# Autodesk Inventor assembly: Robot mrk3
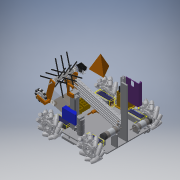
[picture p0: Inventor's stored thumbnail of the model, 180x180]
Saved by Autodesk Inventor 2019 (Build 230136000, 136)
## iProperties
Created: 2017-12-06
Part Number: Robot mrk3
Document SubType Name: Assembly
Designer: User
Author: User
## Documents named in this file (21)
- C:\Robotics\CAD\2018-19_CAD\Robot mrk2.iam
- C:\Robotics\CAD\2017-18_CAD\Prototypes\Gen2PlatePart.ipt
- C:\Robotics\CAD\2017-18_CAD\Prototypes\MecanumWheelFullForVexmotor.iam
- C:\Robotics\CAD\COTSParts\Rev\REV-41-1300HexMotor.ipt
- C:\Robotics\CAD\2017-18_CAD\Prototypes\MotorHolderA.ipt
- C:\Robotics\CAD\2017-18_CAD\Prototypes\MotorHolderB.ipt
- C:\Robotics\CAD\2018-19_CAD\Collection\20X20 lift.iam
- C:\Robotics\CAD\2018-19_CAD\Collection\SlidesPivotBracket.ipt
- C:\Robotics\CAD\2018-19_CAD\Collection\PaddleCollection2.1.ipt.iam
- C:\Robotics\CAD\2018-19_CAD\lift\lift assembly\Lead Screw Prototype A.iam
- C:\Robotics\CAD\2018-19_CAD\Collection\CollectionPost.ipt
- C:\Robotics\CAD\2018-19_CAD\Collection\paddle collection ramp.ipt
- C:\Robotics\CAD\2017-18_CAD\battery for holder.iam
- C:\Robotics\CAD\2018-19_CAD\3d printer\MotoGPhoneHolder.ipt
- C:\Robotics\CAD\COTSParts\Bosch Extrusion\Bosch 20x20 8.5inch.ipt
- C:\Robotics\CAD\COTSParts\Motors\am-3102NeveRest20 (1).ipt
- C:\Robotics\CAD\COTSParts\Actobotics\555 parts\555116ClampingMotorMount37mmBottomBore.ipt
- C:\Robotics\CAD\2018-19_CAD\motor stand.ipt
- C:\Robotics\CAD\2018-19_CAD\3d printer\marker pyramid.ipt
- C:\Robotics\CAD\2018-19_CAD\smart servo with servo block.iam
- PaddleCollection2.1.ipt
## Components (30 placed, 19 different names)
1. Gen2PlatePart:1 — Mate:12, Flush:30, Flush:34, Flush:36, Mate:34, Flush:37, Insert:27, Insert:28, Insert:29, Insert:30, Insert:31, Insert:33, Mate:37, Mate:38, Flush:42, Mate:41, Mate:44, Flush:46, Mate:45, Flush:48, Flush:49, Mate:48, Flush:50, Flush:51, Mate:49, Flush:53, Mate:55, Flush:56, Mate:59, Mate:61, Flush:57, Flush:58, Mate:64
2. MecanumWheelFullForVexmotor:1 [sub-assembly] — Insert:24, Rotation:2, Rotation:3
3. MecanumWheelFullForVexmotor:2 [sub-assembly] — Insert:11, Rotation:1
4. MecanumWheelFullForVexmotor:3 [sub-assembly] — Insert:23, Rotation:1, Rotation:3
5. REV-41-1300HexMotor:2 — Mate:12, Mate:24, Insert:23, Mate:50, Angle:4
6. REV-41-1300HexMotor:3 — Insert:24, Mate:46, Angle:3, Mate:47
7. REV-41-1300HexMotor:4 — Insert:11, Insert:20, Angle:1
8. MotorHolderA:1 — Mate:24, Mate:49, Flush:52, Mate:50, Angle:4
9. MotorHolderA:2 — Flush:30, Insert:25, Mate:45, Flush:48, Flush:49, Angle:2
10. MotorHolderB:1 — Mate:44, Flush:46, Mate:46, Angle:3, Mate:47, Flush:52, Mate:61
11. MotorHolderB:2 — Insert:20, Angle:1, Mate:48, Flush:50, Flush:51
12. REV-41-1300HexMotor:5 — Insert:25, Insert:26, Angle:2
13. MecanumWheelFullForVexmotor:4 [sub-assembly] — Insert:26, Rotation:2
14. SlidesPivotBracket:1 — Mate:31, Insert:27, Insert:28
15. SlidesPivotBracket:2 — Insert:29, Insert:30, Insert:31, Mate:60
16. 20X20 lift:2 [sub-assembly] — Mate:31, Flush:34, Mate:32, Mate:33, Flush:40
17. PaddleCollection2.1.ipt:1 [sub-assembly] — Mate:32, Mate:33, Flush:38, Mate:35, Flush:39, Flush:40
18. Lead Screw Prototype A:1 [sub-assembly] — Mate:34, Flush:37
19. CollectionPost:1 — Insert:33, Flush:53, Mate:56
20. paddle collection ramp:1 — Flush:38, Mate:35, Flush:39
21. battery for holder:1 [sub-assembly] — Mate:37, Mate:38, Flush:42
22. MotoGPhoneHolder:1 — Mate:42, Mate:43, Flush:44
23. Bosch 20x20 8.5inch:1 — Mate:41, Mate:42, Mate:43, Flush:44, Flush:58, Mate:64
24. am-3102NeveRest20 (1):1 — Mate:52, Flush:54
25. am-3102NeveRest20 (1):2 — Mate:51, Flush:55
26. 555116ClampingMotorMount37mmBottomBore:1 — Mate:51, Flush:55, Mate:57, Mate:58
27. 555116ClampingMotorMount37mmBottomBore:2 — Mate:52, Flush:54, Mate:59, Mate:60, Flush:57
28. motor stand:1 — Mate:55, Flush:56, Mate:56, Mate:57, Mate:58
29. smart servo with servo block:1 [sub-assembly]
30. marker pyramid:2
## Relationships (69: Mate 29, Flush 21, Insert 12, Angle 4, RelateRotation 3)
- Mate:12: Gen2PlatePart:1 ↔ REV-41-1300HexMotor:2
- Mate:24: REV-41-1300HexMotor:2 ↔ MotorHolderA:1
- Flush:30: Gen2PlatePart:1 ↔ MotorHolderA:2
- Insert:11: MecanumWheelFullForVexmotor:2 ↔ REV-41-1300HexMotor:4
- Insert:20: REV-41-1300HexMotor:4 ↔ MotorHolderB:2
- Angle:1 (180 deg): REV-41-1300HexMotor:4 ↔ MotorHolderB:2
- Insert:23: MecanumWheelFullForVexmotor:3 ↔ REV-41-1300HexMotor:2
- Insert:24: MecanumWheelFullForVexmotor:1 ↔ REV-41-1300HexMotor:3
- Insert:25: MotorHolderA:2 ↔ REV-41-1300HexMotor:5
- Insert:26: REV-41-1300HexMotor:5 ↔ MecanumWheelFullForVexmotor:4
- Rotation:1 [RelateRotation] (1 ul): MecanumWheelFullForVexmotor:2 ↔ MecanumWheelFullForVexmotor:3
- Rotation:2 [RelateRotation] (1 ul): MecanumWheelFullForVexmotor:1 ↔ MecanumWheelFullForVexmotor:4
- Rotation:3 [RelateRotation] (1 ul): MecanumWheelFullForVexmotor:1 ↔ MecanumWheelFullForVexmotor:3
- Mate:31: SlidesPivotBracket:1 ↔ 20X20 lift:2
- Flush:34 (117.0178 mm): Gen2PlatePart:1 ↔ 20X20 lift:2
- Mate:32: 20X20 lift:2 ↔ PaddleCollection2.1.ipt:1
- Mate:33: 20X20 lift:2 ↔ PaddleCollection2.1.ipt:1
- Flush:36 (360.0704 mm): Gen2PlatePart:1
- Mate:34: Gen2PlatePart:1 ↔ Lead Screw Prototype A:1
- Flush:37: Gen2PlatePart:1 ↔ Lead Screw Prototype A:1
- Insert:27: Gen2PlatePart:1 ↔ SlidesPivotBracket:1
- Insert:28: Gen2PlatePart:1 ↔ SlidesPivotBracket:1
- Insert:29: Gen2PlatePart:1 ↔ SlidesPivotBracket:2
- Insert:30: Gen2PlatePart:1 ↔ SlidesPivotBracket:2
- Insert:31: Gen2PlatePart:1 ↔ SlidesPivotBracket:2
- Insert:33: Gen2PlatePart:1 ↔ CollectionPost:1
- Flush:38: PaddleCollection2.1.ipt:1 ↔ paddle collection ramp:1
- Mate:35: PaddleCollection2.1.ipt:1 ↔ paddle collection ramp:1
- Flush:39 (1.27 mm): PaddleCollection2.1.ipt:1 ↔ paddle collection ramp:1
- Flush:40: 20X20 lift:2 ↔ PaddleCollection2.1.ipt:1
- Mate:37: Gen2PlatePart:1 ↔ battery for holder:1
- Mate:38: Gen2PlatePart:1 ↔ battery for holder:1
- Flush:42: Gen2PlatePart:1 ↔ battery for holder:1
- Mate:41: Gen2PlatePart:1 ↔ Bosch 20x20 8.5inch:1
- Mate:42: MotoGPhoneHolder:1 ↔ Bosch 20x20 8.5inch:1
- Mate:43 (3.048 mm): MotoGPhoneHolder:1 ↔ Bosch 20x20 8.5inch:1
- Flush:44: MotoGPhoneHolder:1 ↔ Bosch 20x20 8.5inch:1
- Mate:44: Gen2PlatePart:1 ↔ MotorHolderB:1
- Flush:46: Gen2PlatePart:1 ↔ MotorHolderB:1
- Mate:45: Gen2PlatePart:1 ↔ MotorHolderA:2
- Flush:48: Gen2PlatePart:1 ↔ MotorHolderA:2
- Flush:49: Gen2PlatePart:1 ↔ MotorHolderA:2
- Angle:2 (180 deg): MotorHolderA:2 ↔ REV-41-1300HexMotor:5
- Mate:46: REV-41-1300HexMotor:3 ↔ MotorHolderB:1
- Angle:3 (180 deg): REV-41-1300HexMotor:3 ↔ MotorHolderB:1
- Mate:47: REV-41-1300HexMotor:3 ↔ MotorHolderB:1
- Mate:48: Gen2PlatePart:1 ↔ MotorHolderB:2
- Flush:50: Gen2PlatePart:1 ↔ MotorHolderB:2
- Flush:51: Gen2PlatePart:1 ↔ MotorHolderB:2
- Mate:49: Gen2PlatePart:1 ↔ MotorHolderA:1
- Flush:52: MotorHolderA:1 ↔ MotorHolderB:1
- Mate:50: REV-41-1300HexMotor:2 ↔ MotorHolderA:1
- Angle:4 (180 deg): REV-41-1300HexMotor:2 ↔ MotorHolderA:1
- Flush:53: Gen2PlatePart:1 ↔ CollectionPost:1
- Mate:51: am-3102NeveRest20 (1):2 ↔ 555116ClampingMotorMount37mmBottomBore:1
- Mate:52: am-3102NeveRest20 (1):1 ↔ 555116ClampingMotorMount37mmBottomBore:2
- Flush:54: am-3102NeveRest20 (1):1 ↔ 555116ClampingMotorMount37mmBottomBore:2
- Flush:55: am-3102NeveRest20 (1):2 ↔ 555116ClampingMotorMount37mmBottomBore:1
- Mate:55: Gen2PlatePart:1 ↔ motor stand:1
- Flush:56 (2.54 mm): Gen2PlatePart:1 ↔ motor stand:1
- Mate:56 (60.96 mm): CollectionPost:1 ↔ motor stand:1
- Mate:57 (-6.35 mm): 555116ClampingMotorMount37mmBottomBore:1 ↔ motor stand:1
- Mate:58: 555116ClampingMotorMount37mmBottomBore:1 ↔ motor stand:1
- Mate:59: Gen2PlatePart:1 ↔ 555116ClampingMotorMount37mmBottomBore:2
- Mate:60 (35.56 mm): SlidesPivotBracket:2 ↔ 555116ClampingMotorMount37mmBottomBore:2
- Mate:61: Gen2PlatePart:1 ↔ MotorHolderB:1
- Flush:57: Gen2PlatePart:1 ↔ 555116ClampingMotorMount37mmBottomBore:2
- Flush:58: Gen2PlatePart:1 ↔ Bosch 20x20 8.5inch:1
- Mate:64 (-6.35 mm): Gen2PlatePart:1 ↔ Bosch 20x20 8.5inch:1
